# Autodesk Inventor assembly: GFRP_T2_12
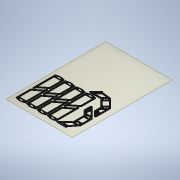
[picture p0: Inventor's stored thumbnail of the model, 180x180]
Saved by Autodesk Inventor 2020 (Build 240168000, 168)
## iProperties
Created: 2021-08-27
Part Number: GFRP_T2_12
Document SubType Name: Assembly
Designer: Masato
Author: Masato
## Documents named in this file (4)
- C:\Inventor\SUSTAINA-OP\Cam\GFRP_T2_12.iam
- C:\Inventor\SUSTAINA-OP\Cam\DisposableBoard.ipt
- C:\Inventor\SUSTAINA-OP\UpperBody\Arm\UpperArm_side_frame.ipt
- C:\Inventor\SUSTAINA-OP\UpperBody\Head\Head_side_frame.ipt
## Components (11 placed, 3 different names)
1. DisposableBoard:1 — メイト:2, メイト:1, フラッシュ:1, フラッシュ:2, フラッシュ:3, メイト:4, メイト:5, フラッシュ:4, メイト:6, メイト:7
2. Head_side_frame:1 — メイト:6, フラッシュ:6, メイト:8, メイト:9
3. Head_side_frame:2 — メイト:7, メイト:9, メイト:10
4. UpperArm_side_frame:1 — メイト:5, フラッシュ:5, 正接:1
5. UpperArm_side_frame:2 — フラッシュ:3, メイト:4, フラッシュ:4, フラッシュ:5, 正接:1
6. UpperArm_side_frame:3
7. UpperArm_side_frame:4
8. UpperArm_side_frame:5
9. UpperArm_side_frame:6
10. UpperArm_side_frame:7 — メイト:10
11. UpperArm_side_frame:8 — フラッシュ:6, メイト:8
## Component patterns: (4 elements, first: UpperArm_side_frame:1 + UpperArm_side_frame:2)
## Relationships (16: Mate 9, Flush 6, Tangent 1)
- メイト:2 [Mate]: DisposableBoard:1
- メイト:1 [Mate]: DisposableBoard:1
- フラッシュ:1 [Flush]: DisposableBoard:1
- フラッシュ:2 [Flush]: DisposableBoard:1
- フラッシュ:3 [Flush] (2 mm): DisposableBoard:1 ↔ UpperArm_side_frame:2
- メイト:4 [Mate]: DisposableBoard:1 ↔ UpperArm_side_frame:2
- メイト:5 [Mate]: DisposableBoard:1 ↔ UpperArm_side_frame:1
- フラッシュ:4 [Flush] (2 mm): DisposableBoard:1 ↔ UpperArm_side_frame:2
- フラッシュ:5 [Flush]: UpperArm_side_frame:1 ↔ UpperArm_side_frame:2
- 正接:1 [Tangent] (2.5 mm): UpperArm_side_frame:1 ↔ UpperArm_side_frame:2
- メイト:6 [Mate]: DisposableBoard:1 ↔ Head_side_frame:1
- メイト:7 [Mate]: DisposableBoard:1 ↔ Head_side_frame:2
- フラッシュ:6 [Flush]: Head_side_frame:1 ↔ UpperArm_side_frame:8
- メイト:8 [Mate] (2.5 mm): Head_side_frame:1 ↔ UpperArm_side_frame:8
- メイト:9 [Mate] (2.5 mm): Head_side_frame:1 ↔ Head_side_frame:2
- メイト:10 [Mate] (2.5 mm): Head_side_frame:2 ↔ UpperArm_side_frame:7
